# Autodesk Inventor assembly: 2in 5mm Hex Stealth Wheel
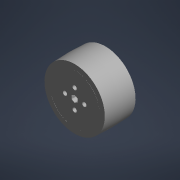
[picture p0: Inventor's stored thumbnail of the model, 180x180]
Saved by Autodesk Inventor 2022 (Build 260153000, 153)
## iProperties
Created: 2019-10-29
Part Number: 2in 5mm Hex Stealth Wheel
Description: STEP AP203
Document SubType Name: Assembly
Designer: izack
Sending System: SolidWorks 2019
Preprocessor: SwSTEP 2.0
Title: am-3664 2in 5mm Hex Bore Stealth Wheel REV2.STEP
Revision Number: ANY
## Documents named in this file (3)
- D:\Robotics\ComputerAidedDesign\2021-22\FTC\#12456 Big Red\Out Take\Elastic Horizontal Rollers\2in 5mm Hex Stealth Wheel.iam
- D:\Robotics\ComputerAidedDesign\2021-22\FTC\Parts\AndyMark\2in Wheel Intergrated 5mm Hex Hub.ipt
- D:\Robotics\ComputerAidedDesign\2021-22\FTC\Parts\AndyMark\2in Tread.ipt
## Components (2 placed, 2 different names)
1. 2in Wheel Intergrated 5mm Hex Hub_1 — Mate:1, Flush:1
2. 2in Tread_2 — Mate:1, Flush:1
## Relationships (2: Mate 1, Flush 1)
- Mate:1: 2in Wheel Intergrated 5mm Hex Hub_1 ↔ 2in Tread_2
- Flush:1: 2in Wheel Intergrated 5mm Hex Hub_1 ↔ 2in Tread_2
